# Autodesk Inventor assembly: temp_hoopSupport
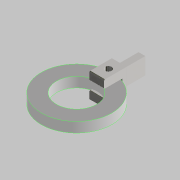
[picture p0: Inventor's stored thumbnail of the model, 180x180]
Saved by Autodesk Inventor 2021 (Build 250183000, 183)
## iProperties
Created: 2021-05-11
Part Number: temp_hoopSupport
Document SubType Name: Assembly
Designer: Watchdog
Author: Watchdog
## Documents named in this file (3)
- C:\Users\Watchdog\OneDrive - Flinders\Advn Mech Design Shared\6_Development\2_Design\inventor\support\temp_hoopSupport.iam
- C:\Users\Watchdog\OneDrive - Flinders\Advn Mech Design Shared\6_Development\2_Design\inventor\support\support_sandwichPlate.ipt
- C:\Users\Watchdog\OneDrive - Flinders\Advn Mech Design Shared\6_Development\2_Design\inventor\support\temp_support_ring.ipt
## Components (2 placed, 2 different names)
1. support_sandwichPlate:1 — Flush:1, Mate:1, Mate:2, Mate:3
2. temp_support_ring:1 — Mate:1
## Relationships (4: Mate 3, Flush 1)
- Flush:1: support_sandwichPlate:1
- Mate:1: support_sandwichPlate:1 ↔ temp_support_ring:1
- Mate:2: support_sandwichPlate:1
- Mate:3: support_sandwichPlate:1
